# Autodesk Inventor assembly: Assembly
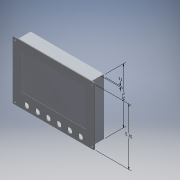
[picture p0: Inventor's stored thumbnail of the model, 180x180]
Saved by Autodesk Inventor 2019 (Build 230136000, 136)
## iProperties
Created: 2021-10-01
Part Number: Assembly
Document SubType Name: Assembly
Designer: maxwe
Author: maxwe
## Documents named in this file (4)
- D:\Makerplane_Efis\EFIS-Hardware-7-inch\New Enclosure\Assembly.iam
- D:\Makerplane_Efis\EFIS-Hardware-7-inch\New Enclosure\NHD-7.ipt
- D:\Makerplane_Efis\EFIS-Hardware-7-inch\New Enclosure\Front Panel.iam
- D:\Makerplane_Efis\EFIS-Hardware-7-inch\New Enclosure\Back Case.ipt
## Components (3 placed, 3 different names)
1. NHD-7:1 — Mate:1, Cylindrical:1, Angle:1, Cylindrical:2
2. Front Panel:1 [sub-assembly] — Mate:1, Cylindrical:1, Angle:1, Angle:2
3. Back Case:1 — Angle:2, Cylindrical:2
## Relationships (5: CylindricalJoint 2, Angle 2, Mate 1)
- Mate:1: NHD-7:1 ↔ Front Panel:1
- Cylindrical:1: NHD-7:1 ↔ Front Panel:1
- Angle:1 (0 deg): NHD-7:1 ↔ Front Panel:1
- Angle:2 (0 deg): Front Panel:1 ↔ Back Case:1
- Cylindrical:2: NHD-7:1 ↔ Back Case:1
